# Autodesk Inventor assembly: LagSamlet
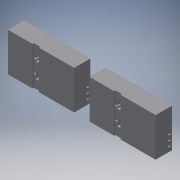
[picture p0: Inventor's stored thumbnail of the model, 180x180]
Saved by Autodesk Inventor 2016 (Build 200138000, 138)
## iProperties
Created: 2016-12-11
Part Number: LagSamlet
Document SubType Name: Assembly
Designer: Simon
Author: Simon
## Documents named in this file (7)
- E:\OneDrive\HTX\Teknologi\YE\LagSamlet.iam
- E:\OneDrive\HTX\Teknologi\YE\Lag1.ipt
- E:\OneDrive\HTX\Teknologi\YE\Lag2.ipt
- E:\OneDrive\HTX\Teknologi\YE\Lag 3.ipt
- E:\OneDrive\HTX\Teknologi\YE\Lag4.ipt
- E:\OneDrive\HTX\Teknologi\YE\Lag5.ipt
- E:\OneDrive\HTX\Teknologi\YE\Lag2-3.ipt
## Components (9 placed, 6 different names)
1. Lag1:2 — Mate:19, Mate:20
2. Lag2-3:1 — Mate:19, Mate:20, Mate:21, Mate:22
3. Lag4:2 — Mate:21, Mate:22, Mate:23, Mate:24
4. Lag5:2 — Mate:23, Mate:24
5. Lag1:1 — Mate:1, Mate:2, Mate:7, Mate:8, Mate:17, Mate:18
6. Lag2:1 — Mate:1, Mate:2, Mate:3, Mate:4, Mate:7, Mate:8, Mate:15, Mate:16, Mate:17, Mate:18
7. Lag 3:1 — Mate:3, Mate:4, Mate:5, Mate:6, Mate:9, Mate:10, Mate:11, Mate:12, Mate:15, Mate:16
8. Lag4:1 — Mate:5, Mate:6, Mate:9, Mate:10, Mate:11, Mate:12, Mate:13, Mate:14
9. Lag5:1 — Mate:13, Mate:14
## Relationships (24: Mate 24)
- Mate:1: Lag1:1 ↔ Lag2:1
- Mate:2: Lag1:1 ↔ Lag2:1
- Mate:3: Lag2:1 ↔ Lag 3:1
- Mate:4: Lag2:1 ↔ Lag 3:1
- Mate:5: Lag 3:1 ↔ Lag4:1
- Mate:6: Lag 3:1 ↔ Lag4:1
- Mate:7: Lag1:1 ↔ Lag2:1
- Mate:8: Lag1:1 ↔ Lag2:1
- Mate:9: Lag 3:1 ↔ Lag4:1
- Mate:10: Lag 3:1 ↔ Lag4:1
- Mate:11: Lag 3:1 ↔ Lag4:1
- Mate:12: Lag 3:1 ↔ Lag4:1
- Mate:13: Lag4:1 ↔ Lag5:1
- Mate:14: Lag4:1 ↔ Lag5:1
- Mate:15: Lag2:1 ↔ Lag 3:1
- Mate:16: Lag2:1 ↔ Lag 3:1
- Mate:17: Lag1:1 ↔ Lag2:1
- Mate:18: Lag1:1 ↔ Lag2:1
- Mate:19: Lag1:2 ↔ Lag2-3:1
- Mate:20: Lag1:2 ↔ Lag2-3:1
- Mate:21: Lag2-3:1 ↔ Lag4:2
- Mate:22: Lag2-3:1 ↔ Lag4:2
- Mate:23: Lag4:2 ↔ Lag5:2
- Mate:24: Lag4:2 ↔ Lag5:2
